# Autodesk Inventor assembly: Assembly1.2
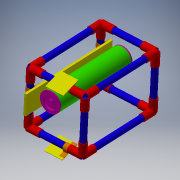
[picture p0: Inventor's stored thumbnail of the model, 180x180]
Saved by Autodesk Inventor 2016 (Build 200138000, 138)
## iProperties
Created: 2017-01-31
Part Number: Assembly1.2
Document SubType Name: Assembly
Designer: student1
Author: student1
## Documents named in this file (9)
- C:\Users\student1\Desktop\Python code\CAD\ROV\OldVersions\Assembly1.2.iam
- C:\Users\student1\Desktop\Python code\CAD\ROV\Frame Part 1.ipt
- C:\Users\student1\Desktop\Python code\CAD\ROV\pvc 1in 3 way elbow noah.ipt
- C:\Users\student1\Desktop\Python code\CAD\ROV\Frame Part 1.5.ipt
- C:\Users\student1\Desktop\Python code\CAD\ROV\Attachy-thing.ipt
- C:\Users\student1\Desktop\Python code\CAD\ROV\Control pipe holder.ipt
- C:\Users\student1\Desktop\Python code\CAD\ROV\motor holder.ipt
- C:\Users\student1\Desktop\Python code\CAD\ROV\O ring Plug 1.ipt
- C:\Users\student1\Desktop\Python code\CAD\ROV\4 inch PVC pipe.ipt
## Components (32 placed, 8 different names)
1. Frame Part 1:1 — Mate:7, Mate:8, Mate:11, Mate:12, Mate:52, Mate:53, Mate:54, Mate:55
2. Frame Part 1:2 — Mate:3, Mate:4, Mate:9, Mate:10
3. Frame Part 1:3 — Mate:1, Mate:2, Mate:5, Mate:6
4. Frame Part 1:4 — Mate:13, Mate:14, Mate:15, Mate:16
5. pvc 1in 3 way elbow noah:1 — Mate:1, Mate:2, Mate:3, Mate:4, Mate:18, Mate:22
6. pvc 1in 3 way elbow noah:2 — Mate:5, Mate:6, Mate:7, Mate:8, Mate:17, Mate:21
7. pvc 1in 3 way elbow noah:3 — Mate:11, Mate:12, Mate:13, Mate:15, Mate:20, Mate:24, Mate:83
8. pvc 1in 3 way elbow noah:4 — Mate:9, Mate:10, Mate:14, Mate:16, Mate:19, Mate:23
9. Frame Part 1.5:1 — Mate:17, Mate:21, Mate:26, Mate:27, Mate:31
10. Frame Part 1.5:2 — Mate:18, Mate:22, Mate:29, Mate:32
11. Frame Part 1.5:3 — Mate:20, Mate:24, Mate:25, Mate:28
12. Frame Part 1.5:4 — Mate:19, Mate:23, Mate:30, Mate:33
13. pvc 1in 3 way elbow noah:5 — Mate:26, Mate:27, Mate:31, Mate:35, Mate:37, Mate:46
14. pvc 1in 3 way elbow noah:6 — Mate:25, Mate:28, Mate:39, Mate:41, Mate:43, Mate:45
15. pvc 1in 3 way elbow noah:7 — Mate:30, Mate:33, Mate:38, Mate:40, Mate:42, Mate:44, Mate:70
16. pvc 1in 3 way elbow noah:8 — Mate:29, Mate:32, Mate:34, Mate:36, Mate:47, Mate:71
17. Frame Part 1:5 — Mate:43, Mate:45, Mate:46, Mate:48, Mate:49, Mate:50, Mate:51
18. Frame Part 1:6 — Mate:42, Mate:44, Mate:47
19. Frame Part 1:7 — Mate:38, Mate:39, Mate:40, Mate:41, Mate:68, Mate:69
20. Frame Part 1:8 — Mate:34, Mate:35, Mate:36, Mate:37, Mate:66, Mate:67
21. Attachy-thing:1 — Mate:50, Mate:51, Mate:56, Mate:63
22. Attachy-thing:2 — Mate:48, Mate:49, Mate:57, Mate:60
23. Attachy-thing:3 — Mate:52, Mate:53, Mate:59, Mate:61, Mate:64
24. Attachy-thing:4 — Mate:54, Mate:55, Mate:58, Mate:62, Mate:65, Mate:83
25. Control pipe holder:1 — Mate:56, Mate:57, Mate:58, Mate:59, Mate:60, Mate:61, Mate:62, Mate:63, Mate:64, Mate:65, Tangent:1, Mate:82
26. Attachy-thing:5 — Mate:66, Mate:67, Mate:71, Mate:72, Mate:73, Mate:74
27. Attachy-thing:6 — Mate:68, Mate:69, Mate:70, Mate:75, Mate:76, Mate:77
28. motor holder:1 — Mate:72, Mate:73, Mate:74, Mate:84
29. motor holder:2 — Mate:75, Mate:76, Mate:77, Mate:84
30. O ring Plug 1:1 — Mate:80, Mate:81, Mate:82
31. O ring Plug 1:2 — Mate:78, Mate:79
32. 4 inch PVC pipe:1 — Mate:78, Mate:79, Mate:80, Mate:81, Tangent:1
## Relationships (85: Mate 84, Tangent 1)
- Mate:1: Frame Part 1:3 ↔ pvc 1in 3 way elbow noah:1
- Mate:2: Frame Part 1:3 ↔ pvc 1in 3 way elbow noah:1
- Mate:3: Frame Part 1:2 ↔ pvc 1in 3 way elbow noah:1
- Mate:4: Frame Part 1:2 ↔ pvc 1in 3 way elbow noah:1
- Mate:5: Frame Part 1:3 ↔ pvc 1in 3 way elbow noah:2
- Mate:6: Frame Part 1:3 ↔ pvc 1in 3 way elbow noah:2
- Mate:7: Frame Part 1:1 ↔ pvc 1in 3 way elbow noah:2
- Mate:8: Frame Part 1:1 ↔ pvc 1in 3 way elbow noah:2
- Mate:9: Frame Part 1:2 ↔ pvc 1in 3 way elbow noah:4
- Mate:10: Frame Part 1:2 ↔ pvc 1in 3 way elbow noah:4
- Mate:11: Frame Part 1:1 ↔ pvc 1in 3 way elbow noah:3
- Mate:12: Frame Part 1:1 ↔ pvc 1in 3 way elbow noah:3
- Mate:13: Frame Part 1:4 ↔ pvc 1in 3 way elbow noah:3
- Mate:14: Frame Part 1:4 ↔ pvc 1in 3 way elbow noah:4
- Mate:15: Frame Part 1:4 ↔ pvc 1in 3 way elbow noah:3
- Mate:16: Frame Part 1:4 ↔ pvc 1in 3 way elbow noah:4
- Mate:17: pvc 1in 3 way elbow noah:2 ↔ Frame Part 1.5:1
- Mate:18: pvc 1in 3 way elbow noah:1 ↔ Frame Part 1.5:2
- Mate:19: pvc 1in 3 way elbow noah:4 ↔ Frame Part 1.5:4
- Mate:20: pvc 1in 3 way elbow noah:3 ↔ Frame Part 1.5:3
- Mate:21: pvc 1in 3 way elbow noah:2 ↔ Frame Part 1.5:1
- Mate:22: pvc 1in 3 way elbow noah:1 ↔ Frame Part 1.5:2
- Mate:23: pvc 1in 3 way elbow noah:4 ↔ Frame Part 1.5:4
- Mate:24: pvc 1in 3 way elbow noah:3 ↔ Frame Part 1.5:3
- Mate:25: Frame Part 1.5:3 ↔ pvc 1in 3 way elbow noah:6
- Mate:26: Frame Part 1.5:1 ↔ pvc 1in 3 way elbow noah:5
- Mate:27: Frame Part 1.5:1 ↔ pvc 1in 3 way elbow noah:5
- Mate:28: Frame Part 1.5:3 ↔ pvc 1in 3 way elbow noah:6
- Mate:29: Frame Part 1.5:2 ↔ pvc 1in 3 way elbow noah:8
- Mate:30: Frame Part 1.5:4 ↔ pvc 1in 3 way elbow noah:7
- Mate:31: Frame Part 1.5:1 ↔ pvc 1in 3 way elbow noah:5
- Mate:32: Frame Part 1.5:2 ↔ pvc 1in 3 way elbow noah:8
- Mate:33: Frame Part 1.5:4 ↔ pvc 1in 3 way elbow noah:7
- Mate:34: pvc 1in 3 way elbow noah:8 ↔ Frame Part 1:8
- Mate:35: pvc 1in 3 way elbow noah:5 ↔ Frame Part 1:8
- Mate:36: pvc 1in 3 way elbow noah:8 ↔ Frame Part 1:8
- Mate:37: pvc 1in 3 way elbow noah:5 ↔ Frame Part 1:8
- Mate:38: pvc 1in 3 way elbow noah:7 ↔ Frame Part 1:7
- Mate:39: pvc 1in 3 way elbow noah:6 ↔ Frame Part 1:7
- Mate:40: pvc 1in 3 way elbow noah:7 ↔ Frame Part 1:7
- Mate:41: pvc 1in 3 way elbow noah:6 ↔ Frame Part 1:7
- Mate:42: pvc 1in 3 way elbow noah:7 ↔ Frame Part 1:6
- Mate:43: pvc 1in 3 way elbow noah:6 ↔ Frame Part 1:5
- Mate:44: pvc 1in 3 way elbow noah:7 ↔ Frame Part 1:6
- Mate:45: pvc 1in 3 way elbow noah:6 ↔ Frame Part 1:5
- Mate:46: pvc 1in 3 way elbow noah:5 ↔ Frame Part 1:5
- Mate:47: pvc 1in 3 way elbow noah:8 ↔ Frame Part 1:6
- Mate:48: Frame Part 1:5 ↔ Attachy-thing:2
- Mate:49: Frame Part 1:5 ↔ Attachy-thing:2
- Mate:50: Frame Part 1:5 ↔ Attachy-thing:1
- Mate:51: Frame Part 1:5 ↔ Attachy-thing:1
- Mate:52: Frame Part 1:1 ↔ Attachy-thing:3
- Mate:53: Frame Part 1:1 ↔ Attachy-thing:3
- Mate:54: Frame Part 1:1 ↔ Attachy-thing:4
- Mate:55: Frame Part 1:1 ↔ Attachy-thing:4
- Mate:56: Attachy-thing:1 ↔ Control pipe holder:1
- Mate:57: Attachy-thing:2 ↔ Control pipe holder:1
- Mate:58: Attachy-thing:4 ↔ Control pipe holder:1
- Mate:59: Attachy-thing:3 ↔ Control pipe holder:1
- Mate:60: Attachy-thing:2 ↔ Control pipe holder:1
- Mate:61: Attachy-thing:3 ↔ Control pipe holder:1
- Mate:62: Attachy-thing:4 ↔ Control pipe holder:1
- Mate:63: Attachy-thing:1 ↔ Control pipe holder:1
- Mate:64: Attachy-thing:3 ↔ Control pipe holder:1
- Mate:65: Attachy-thing:4 ↔ Control pipe holder:1
- Mate:66: Frame Part 1:8 ↔ Attachy-thing:5
- Mate:67: Frame Part 1:8 ↔ Attachy-thing:5
- Mate:68: Frame Part 1:7 ↔ Attachy-thing:6
- Mate:69: Frame Part 1:7 ↔ Attachy-thing:6
- Mate:70: pvc 1in 3 way elbow noah:7 ↔ Attachy-thing:6
- Mate:71: pvc 1in 3 way elbow noah:8 ↔ Attachy-thing:5
- Mate:72: Attachy-thing:5 ↔ motor holder:1
- Mate:73: Attachy-thing:5 ↔ motor holder:1
- Mate:74: Attachy-thing:5 ↔ motor holder:1
- Mate:75: Attachy-thing:6 ↔ motor holder:2
- Mate:76: Attachy-thing:6 ↔ motor holder:2
- Mate:77: Attachy-thing:6 ↔ motor holder:2
- Mate:78: O ring Plug 1:2 ↔ 4 inch PVC pipe:1
- Mate:79: O ring Plug 1:2 ↔ 4 inch PVC pipe:1
- Mate:80: O ring Plug 1:1 ↔ 4 inch PVC pipe:1
- Mate:81: O ring Plug 1:1 ↔ 4 inch PVC pipe:1
- Tangent:1: Control pipe holder:1 ↔ 4 inch PVC pipe:1
- Mate:82: Control pipe holder:1 ↔ O ring Plug 1:1
- Mate:83 (25.4 mm): pvc 1in 3 way elbow noah:3 ↔ Attachy-thing:4
- Mate:84: motor holder:1 ↔ motor holder:2
